# Autodesk Inventor assembly: IMU Assembly
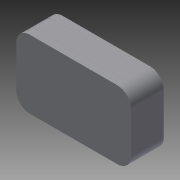
[picture p0: Inventor's stored thumbnail of the model, 180x180]
Saved by Autodesk Inventor 2015 (Build 190159000, 159)
## iProperties
Created: 2015-05-29
Part Number: IMU Assembly
Document SubType Name: Assembly
Designer: Evil Brian
Author: Evil Brian
## Documents named in this file (4)
- C:\Users\Evil Brian\Documents\CAD Temporary Files for GitHub Upload\IMU Assembly.iam
- C:\Users\Evil Brian\Documents\CAD Temporary Files for GitHub Upload\IMU Bottom 3mm.ipt
- C:\Users\Evil Brian\Documents\CAD Temporary Files for GitHub Upload\IMU Center 6mm.ipt
- C:\Users\Evil Brian\Documents\CAD Temporary Files for GitHub Upload\IMU Top 3mm.ipt
## Components (3 placed, 3 different names)
1. IMU Bottom 3mm:1 — Mate:1, Flush:1, Flush:2, Flush:3, Flush:4
2. IMU Center 6mm:1 — Mate:1, Flush:1, Flush:2, Mate:2
3. IMU Top 3mm:1 — Mate:2, Flush:3, Flush:4
## Relationships (6: Flush 4, Mate 2)
- Mate:1: IMU Bottom 3mm:1 ↔ IMU Center 6mm:1
- Flush:1: IMU Bottom 3mm:1 ↔ IMU Center 6mm:1
- Flush:2: IMU Bottom 3mm:1 ↔ IMU Center 6mm:1
- Mate:2: IMU Center 6mm:1 ↔ IMU Top 3mm:1
- Flush:3: IMU Bottom 3mm:1 ↔ IMU Top 3mm:1
- Flush:4: IMU Bottom 3mm:1 ↔ IMU Top 3mm:1
